# Autodesk Inventor assembly: zlozenie_Z
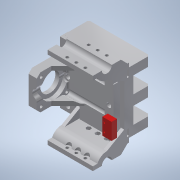
[picture p0: Inventor's stored thumbnail of the model, 180x180]
Saved by Autodesk Inventor 2020 (Build 240168000, 168)
## iProperties
Created: 2020-08-11
Part Number: zlozenie_Z
Material: Ogólny
Document SubType Name: Assembly
Designer: invin
Mass: 196.401 g
Surface Area: 751.475 cm^2
Volume: 185.284 cm^3
Density: 1.06 g/cm^3
Author: invin
## Documents named in this file (6)
- D:\KONIECTEGOKOŁCHOZU\MGR\Model\Workspaces\Obszar roboczy\assembly_v3\Y\YSub1.iam
- D:\KONIECTEGOKOŁCHOZU\MGR\Model\Workspaces\Obszar roboczy\content\manipulatorSharedParts\stopSw.ipt
- D:\KONIECTEGOKOŁCHOZU\MGR\Model\Workspaces\Obszar roboczy\assembly_v3\Y\YItemEnd.ipt
- D:\KONIECTEGOKOŁCHOZU\MGR\Model\Workspaces\Obszar roboczy\assembly_v3\Y\YEndStopMount.ipt
- D:\KONIECTEGOKOŁCHOZU\MGR\Model\Workspaces\Obszar roboczy\assembly_v3\Y\YMotorMount.ipt
- D:\KONIECTEGOKOŁCHOZU\MGR\Model\Workspaces\Obszar roboczy\assembly_v3\Y\YRodMount.ipt
## Components (5 placed, 5 different names)
1. YItemEnd:1 — Zestawiający:4, Zestawiający:5, Zestawiający:12, Równoległe:1, Równoległe:2, Zestawiające:13
2. YRodMount:1 — Zestawiający:4, Zestawiający:5, Zestawiający:9, Zestawiający:10, Zestawiający:11, Zestawiający:12
3. YMotorMount:1 — Zestawiający:9, Zestawiający:10, Zestawiający:11, Zestawiające:14, Zestawiające:15, Zestawiające:16
4. YEndStopMount:1 — Zestawiające:14, Zestawiające:15, Zestawiające:16, Zestawiające:17, Zestawiające:18, Zestawiające:19
5. stopSw:1 — Zestawiające:17, Zestawiające:18, Zestawiające:19
## Relationships (15: Mate 13, Flush 2)
- Zestawiający:4 [Mate]: YItemEnd:1 ↔ YRodMount:1
- Zestawiający:5 [Mate]: YItemEnd:1 ↔ YRodMount:1
- Zestawiający:9 [Mate]: YRodMount:1 ↔ YMotorMount:1
- Zestawiający:10 [Mate]: YRodMount:1 ↔ YMotorMount:1
- Zestawiający:11 [Mate]: YRodMount:1 ↔ YMotorMount:1
- Zestawiający:12 [Mate]: YItemEnd:1 ↔ YRodMount:1
- Równoległe:1 [Flush]: YItemEnd:1
- Równoległe:2 [Flush]: YItemEnd:1
- Zestawiające:13 [Mate]: YItemEnd:1
- Zestawiające:14 [Mate]: YMotorMount:1 ↔ YEndStopMount:1
- Zestawiające:15 [Mate]: YMotorMount:1 ↔ YEndStopMount:1
- Zestawiające:16 [Mate]: YMotorMount:1 ↔ YEndStopMount:1
- Zestawiające:17 [Mate]: YEndStopMount:1 ↔ stopSw:1
- Zestawiające:18 [Mate]: YEndStopMount:1 ↔ stopSw:1
- Zestawiające:19 [Mate]: YEndStopMount:1 ↔ stopSw:1
